# Autodesk Inventor assembly: J007251
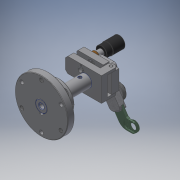
[picture p0: Inventor's stored thumbnail of the model, 180x180]
Saved by Autodesk Inventor 2018.2 (Build 222227000, 227)
## iProperties
Created: 2016-09-01
Vendor: HHMI: JRC - ID&F
Document SubType Name: Assembly
Designer: ARNOLDJ
Part Number: J007251
Description: LFOV TILT STAGE
RuleStatus: InUse
AfterDocSave0: file://Part Number Cleaner
DESIGN DEPARTMENT: HHMI: JRC - ID&F
ALTERED ITEM PART NUMBER: N/A
ALTERED ITEM VENDOR: N/A
ALTERED ITEM DESCRIPTION: N/A
Revision Number: 0
## Documents named in this file (17)
- C:\_WORKSPACE\DATA\PROJECTS\_PROJECTS BY LAB\HANTMAN (LAB)\LFOV TILT STAGE\LFOV TILT STAGE.iam
- C:\_WORKSPACE\DATA\PROJECTS\MOUSE FOOD DELIVERY AND JOY STICK SYSTEM\MCAD\ANGLE ADJ LOWER.ipt
- C:\_WORKSPACE\DATA\PROJECTS\MOUSE FOOD DELIVERY AND JOY STICK SYSTEM\MCAD\ANGLE ADJ UPPER.ipt
- C:\_WORKSPACE\DATA\PROJECTS\MOUSE FOOD DELIVERY AND JOY STICK SYSTEM\MCAD\F25SSN2P.ipt
- C:\_WORKSPACE\DATA\PROJECTS\MOUSE FOOD DELIVERY AND JOY STICK SYSTEM\MCAD\FAS100.ipt
- C:\_WORKSPACE\DATA\PROJECTS\MOUSE FOOD DELIVERY AND JOY STICK SYSTEM\MCAD\MBS CLAMP ARM TRAINER.ipt
- C:\_WORKSPACE\DATA\PROJECTS\MOUSE FOOD DELIVERY AND JOY STICK SYSTEM\MCAD\TR2 AI.ipt
- C:\_WORKSPACE\DATA\PROJECTS\MOUSE FOOD DELIVERY AND JOY STICK SYSTEM\MCAD\90145A417.ipt
- C:\_WORKSPACE\DATA\PROJECTS\MOUSE FOOD DELIVERY AND JOY STICK SYSTEM\MCAD\90145A475.ipt
- C:\_WORKSPACE\DATA\PROJECTS\_PROJECTS BY LAB\SVOBODA (LAB)\MOUSE POSITIONING SYSTEMS\MCAD\BALL SETUP\MBS POS-T-SCREW.iam
- C:\_WORKSPACE\DATA\PROJECTS\MOUSE FOOD DELIVERY AND JOY STICK SYSTEM\MCAD\93475A240.ipt
- C:\_WORKSPACE\DATA\PROJECTS\MOUSE FOOD DELIVERY AND JOY STICK SYSTEM\MCAD\91292A125.ipt
- C:\_WORKSPACE\DATA\PROJECTS\_PROJECTS BY LAB\HANTMAN (LAB)\LFOV TILT STAGE\9793T130.ipt
- C:\_WORKSPACE\DATA\PROJECTS\_PROJECTS BY LAB\SVOBODA (LAB)\MOUSE POSITIONING SYSTEMS\MCAD\BALL SETUP\MBS INLINE RING TAB.ipt
- C:\_WORKSPACE\DATA\PROJECTS\_PROJECTS BY LAB\SVOBODA (LAB)\MOUSE POSITIONING SYSTEMS\MCAD\BALL SETUP\MBS CLAMP PLATE.ipt
- C:\_WORKSPACE\DATA\PROJECTS\MOUSE FOOD DELIVERY AND JOY STICK SYSTEM\MCAD\92185A192.ipt
- C:\_WORKSPACE\DATA\PROJECTS\MOUSE FOOD DELIVERY AND JOY STICK SYSTEM\MCAD\B3-11.ipt
## Components (22 placed, 16 different names)
1. ANGLE ADJ LOWER:1 — Mate:1, Mate:2, Mate:3, Mate:4, Angle:1, Mate:16, Tangent:8, Tangent:9, Mate:21, Flush:3, Mate:36, Mate:37
2. TR2 AI:1 — Mate:1, Mate:2, Flush:4, Mate:30
3. ANGLE ADJ UPPER:1 — Mate:3, Mate:4, Angle:1, Mate:9, Mate:10, Mate:11, Angle:2, Mate:14, Mate:15, Tangent:6, Tangent:7, Mate:18, Mate:27
4. F25SSN2P:1 — Flush:1, Mate:7, Mate:9, Mate:14
5. FAS100:1 — Flush:1, Mate:7
6. MBS CLAMP ARM TRAINER:1 — Mate:10, Mate:11, Angle:2, Mate:25, Mate:26, Mate:31, Mate:32, Tangent:10, Mate:33, Mate:34, Angle:4
7. 90145A417:5
8. 90145A417:6
9. 90145A475:1 — Mate:21, Flush:3
10. MBS POS-T-SCREW:1 [sub-assembly] — Mate:25, Mate:35
11. 93475A240:1 — Mate:26, Mate:27, Mate:28, Mate:29
12. 91292A125:1 — Mate:28, Mate:29
13. 9793T130:1 — Flush:4, Mate:30
14. MBS INLINE RING TAB:1 — Mate:31, Mate:32, Tangent:10
15. MBS CLAMP PLATE:1 — Mate:33, Mate:34, Angle:4, Mate:35
16. 92185A192:1 — Mate:36, Mate:37
17. 90145A417:1 — Mate:15, Tangent:6, Tangent:7, Mate:17, Angle:3, Mate:19, Mate:20
18. B3-11:1 — Mate:17, Mate:18, Angle:3, Mate:19, Mate:20
19. 90145A417:2 — Mate:16, Tangent:8, Tangent:9
20. 90145A417:3
21. B3-11:2
22. 90145A417:4
## Component patterns: (2 elements, first: 90145A417:1 + B3-11:1 + 90145A417:2)
## Relationships (49: Mate 31, Tangent 10, Flush 4, Angle 4)
- Mate:1: ANGLE ADJ LOWER:1 ↔ TR2 AI:1
- Mate:2: ANGLE ADJ LOWER:1 ↔ TR2 AI:1
- Mate:3: ANGLE ADJ LOWER:1 ↔ ANGLE ADJ UPPER:1
- Mate:4: ANGLE ADJ LOWER:1 ↔ ANGLE ADJ UPPER:1
- Flush:1: F25SSN2P:1 ↔ FAS100:1
- Mate:7: F25SSN2P:1 ↔ FAS100:1
- Angle:1 (0 deg): ANGLE ADJ LOWER:1 ↔ ANGLE ADJ UPPER:1
- Mate:9: ANGLE ADJ UPPER:1 ↔ F25SSN2P:1
- Mate:10: ANGLE ADJ UPPER:1 ↔ MBS CLAMP ARM TRAINER:1
- Mate:11: ANGLE ADJ UPPER:1 ↔ MBS CLAMP ARM TRAINER:1
- Angle:2 (0 deg): ANGLE ADJ UPPER:1 ↔ MBS CLAMP ARM TRAINER:1
- [Mate]: ANGLE ADJ LOWER:1 ↔ 90145A417:6
- [Tangent]: ANGLE ADJ LOWER:1 ↔ 90145A417:6
- [Tangent]: ANGLE ADJ LOWER:1 ↔ 90145A417:6
- [Mate]: ANGLE ADJ LOWER:1 ↔ 90145A417:5
- [Tangent]: ANGLE ADJ LOWER:1 ↔ 90145A417:5
- [Tangent]: ANGLE ADJ LOWER:1 ↔ 90145A417:5
- [Tangent]: FAS100:1 ↔ 90145A417:5
- Mate:14: ANGLE ADJ UPPER:1 ↔ F25SSN2P:1
- Mate:15 (0.381 mm): ANGLE ADJ UPPER:1 ↔ 90145A417:1
- Tangent:6 (0.0381 mm): ANGLE ADJ UPPER:1 ↔ 90145A417:1
- Tangent:7: ANGLE ADJ UPPER:1 ↔ 90145A417:1
- Mate:16 (0.381 mm): ANGLE ADJ LOWER:1 ↔ 90145A417:2
- Tangent:8: ANGLE ADJ LOWER:1 ↔ 90145A417:2
- Tangent:9 (0.0889 mm): ANGLE ADJ LOWER:1 ↔ 90145A417:2
- Flush:2 (6.35 mm)
- Mate:17: 90145A417:1 ↔ B3-11:1
- Mate:18: ANGLE ADJ UPPER:1 ↔ B3-11:1
- Angle:3 (0 deg): 90145A417:1 ↔ B3-11:1
- Mate:19: 90145A417:1 ↔ B3-11:1
- Mate:20: 90145A417:1 ↔ B3-11:1
- Mate:21: ANGLE ADJ LOWER:1 ↔ 90145A475:1
- Flush:3: ANGLE ADJ LOWER:1 ↔ 90145A475:1
- Mate:25: MBS CLAMP ARM TRAINER:1 ↔ MBS POS-T-SCREW:1
- Mate:26: MBS CLAMP ARM TRAINER:1 ↔ 93475A240:1
- Mate:27: ANGLE ADJ UPPER:1 ↔ 93475A240:1
- Mate:28: 93475A240:1 ↔ 91292A125:1
- Mate:29: 93475A240:1 ↔ 91292A125:1
- Flush:4: TR2 AI:1 ↔ 9793T130:1
- Mate:30: TR2 AI:1 ↔ 9793T130:1
- Mate:31: MBS CLAMP ARM TRAINER:1 ↔ MBS INLINE RING TAB:1
- Mate:32: MBS CLAMP ARM TRAINER:1 ↔ MBS INLINE RING TAB:1
- Tangent:10: MBS CLAMP ARM TRAINER:1 ↔ MBS INLINE RING TAB:1
- Mate:33: MBS CLAMP ARM TRAINER:1 ↔ MBS CLAMP PLATE:1
- Mate:34: MBS CLAMP ARM TRAINER:1 ↔ MBS CLAMP PLATE:1
- Angle:4 (0 deg): MBS CLAMP ARM TRAINER:1 ↔ MBS CLAMP PLATE:1
- Mate:35: MBS POS-T-SCREW:1 ↔ MBS CLAMP PLATE:1
- Mate:36: ANGLE ADJ LOWER:1 ↔ 92185A192:1
- Mate:37: ANGLE ADJ LOWER:1 ↔ 92185A192:1
